# Autodesk Inventor assembly: Assembly1
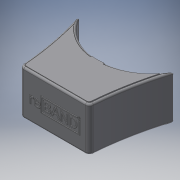
[picture p0: Inventor's stored thumbnail of the model, 180x180]
Saved by Autodesk Inventor 2018 (Build 220112000, 112)
## iProperties
Created: 2020-07-06
Part Number: Assembly1
Document SubType Name: Assembly
Designer: maqur
Author: maqur
## Documents named in this file (4)
- C:\Users\maqur\Documents\reBAND CAD\Assembly1.iam
- C:\Users\maqur\Documents\headset.ipt
- C:\Users\maqur\Documents\reBAND CAD\ArduinoModule.ipt
- C:\Users\maqur\Documents\reBAND CAD\headset cover.ipt
## Components (3 placed, 3 different names)
1. headset:1 — Mate:1, Mate:2, Mate:3, Mate:4, Mate:5, Mate:6
2. ArduinoModule:1 — Mate:1, Mate:2, Mate:3
3. headset cover:1 — Mate:4, Mate:5, Mate:6
## Relationships (6: Mate 6)
- Mate:1: headset:1 ↔ ArduinoModule:1
- Mate:2: headset:1 ↔ ArduinoModule:1
- Mate:3: headset:1 ↔ ArduinoModule:1
- Mate:4: headset:1 ↔ headset cover:1
- Mate:5: headset:1 ↔ headset cover:1
- Mate:6: headset:1 ↔ headset cover:1
